# Autodesk Inventor assembly: Assembly of moving unit MY ADDITION
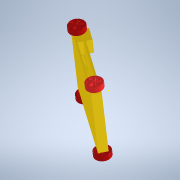
[picture p0: Inventor's stored thumbnail of the model, 180x180]
Saved by Autodesk Inventor 2021 (Build 250183000, 183)
## iProperties
Created: 2021-07-07
Part Number: Assembly of moving unit MY ADDITION
Document SubType Name: Assembly
Designer: AKSHATA
Author: AKSHATA
## Documents named in this file (4)
- C:\Users\HP\Downloads\Assembly of moving unit MY ADDITION.iam
- C:\Users\HP\Downloads\BASE7.ipt
- C:\Users\AKSHATA\Documents\WHEEL AXLE2.ipt
- C:\Users\HP\Downloads\WHEEL 2.ipt
## Components (7 placed, 3 different names)
1. BASE7:1 — Mate:1, Mate:2, Mate:3, Mate:4, Mate:6, Mate:8, Mate:10, Mate:12
2. WHEEL AXLE2:1 — Mate:1, Mate:2, Mate:5, Mate:9
3. WHEEL AXLE2:2 — Mate:3, Mate:4, Mate:7, Mate:11
4. WHEEL 2:1 — Mate:5, Mate:6
5. WHEEL 2:2 — Mate:7, Mate:8
6. WHEEL 2:4 — Mate:9, Mate:10
7. WHEEL 2:5 — Mate:11, Mate:12
## Relationships (12: Mate 12)
- Mate:1: BASE7:1 ↔ WHEEL AXLE2:1
- Mate:2 (20 mm): BASE7:1 ↔ WHEEL AXLE2:1
- Mate:3: BASE7:1 ↔ WHEEL AXLE2:2
- Mate:4 (20 mm): BASE7:1 ↔ WHEEL AXLE2:2
- Mate:5: WHEEL AXLE2:1 ↔ WHEEL 2:1
- Mate:6 (5 mm): BASE7:1 ↔ WHEEL 2:1
- Mate:7: WHEEL AXLE2:2 ↔ WHEEL 2:2
- Mate:8 (5 mm): BASE7:1 ↔ WHEEL 2:2
- Mate:9: WHEEL AXLE2:1 ↔ WHEEL 2:4
- Mate:10 (5 mm): BASE7:1 ↔ WHEEL 2:4
- Mate:11: WHEEL AXLE2:2 ↔ WHEEL 2:5
- Mate:12 (5 mm): BASE7:1 ↔ WHEEL 2:5
